# Autodesk Inventor assembly: actuMount
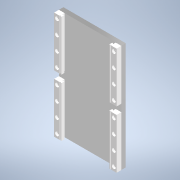
[picture p0: Inventor's stored thumbnail of the model, 180x180]
Saved by Autodesk Inventor 2021 (Build 250183000, 183)
## iProperties
Created: 2021-03-29
Part Number: actuMount
Document SubType Name: Assembly
Designer: Work
Author: Work
## Documents named in this file (3)
- C:\Users\Work\OneDrive - Brookhaven National Laboratory\Daniels, William intern HPR station\Frame\actuMount.iam
- C:\Users\Work\OneDrive - Brookhaven National Laboratory\Daniels, William intern HPR station\Frame\actuPlate.ipt
- C:\Users\Work\OneDrive - Brookhaven National Laboratory\Daniels, William intern HPR station\Frame\actuClip.ipt
## Components (5 placed, 2 different names)
1. actuPlate:1 — Rotational:1, Rotational:2, Rigid:1, Rigid:2
2. actuClip:1 — Rotational:1
3. actuClip:2 — Rotational:2
4. actuClip:3 — Rigid:1
5. actuClip:4 — Rigid:2
## Relationships (4: RevoluteJoint 2, WeldJoint 2)
- Rotational:1 [RevoluteJoint]: actuPlate:1 ↔ actuClip:1
- Rotational:2 [RevoluteJoint]: actuPlate:1 ↔ actuClip:2
- Rigid:1 [WeldJoint]: actuPlate:1 ↔ actuClip:3
- Rigid:2 [WeldJoint]: actuPlate:1 ↔ actuClip:4
